# Autodesk Inventor assembly: LinearBearingPlusClamps
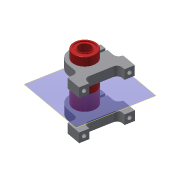
[picture p0: Inventor's stored thumbnail of the model, 180x180]
Saved by Autodesk Inventor 2018 (Build 220112000, 112)
## iProperties
Created: 2017-12-09
Part Number: LinearBearingPlusClamps
Document SubType Name: Assembly
Designer: ball
Author: ball
## Documents named in this file (3)
- C:\FTC\FTC8863CAD\2017Robot\LinearBearingPlusClamps.iam
- C:\FTC\FTC8863CAD\Actobotics\535 parts\535226.ipt
- C:\FTC\FTC8863CAD\Actobotics\585 parts\585640.ipt
## Components (3 placed, 2 different names)
1. 535226:1
2. 585640:1 — Angle:1, Angle:2, Mate:2, Symmetry:1
3. 585640:2 — Angle:1, Angle:2, Mate:2, Symmetry:1
## Relationships (6: Mate 2, Angle 2, Flush 1, Symmetry 1)
- [Mate]: 535226:1 ↔ 585640:1
- [Flush] (5.7912 mm): 535226:1 ↔ 585640:1
- Angle:1 (0 deg): 585640:1 ↔ 585640:2
- Angle:2 (0 deg): 585640:1 ↔ 585640:2
- Mate:2 (-26.9494 mm): 585640:1 ↔ 585640:2
- Symmetry:1: 585640:1 ↔ 585640:2
